# Autodesk Inventor assembly: Connector Box
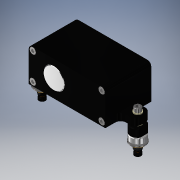
[picture p0: Inventor's stored thumbnail of the model, 180x180]
Saved by Autodesk Inventor 2019 (Build 230136000, 136)
## iProperties
Created: 2018-05-06
Part Number: Connector Box
Document SubType Name: Assembly
Designer: IEUser
Author: IEUser
## Documents named in this file (11)
- C:\Users\IEUser\Desktop\lrut-inflatable-ring-standard-master\Connector Box\Connector Box.iam
- C:\Users\IEUser\Desktop\lrut-inflatable-ring-standard-master\Connector Box\Connector Lid.ipt
- C:\Users\IEUser\Desktop\lrut-inflatable-ring-standard-master\Stock Components\LEMO\73397830-9-egg_4b_324_cll\egg_4b_324_cll_01.ipt
- C:\Users\IEUser\Desktop\lrut-inflatable-ring-standard-master\Stock Components\LEMO\73397830-9-egg_4b_324_cll\egg_4b_324_cll_02.ipt
- C:\Users\IEUser\Desktop\lrut-inflatable-ring-standard-master\Stock Components\LEMO\73397830-9-egg_4b_324_cll\egg_4b_324_cll_03.ipt
- C:\Users\IEUser\Desktop\lrut-inflatable-ring-standard-master\Connector Box\Connector Box.ipt
- C:\Users\IEUser\Desktop\lrut-inflatable-ring-standard-master\Stock Components\Accu Group\SSCF-M5-10-A4.ipt
- C:\Users\IEUser\Desktop\lrut-inflatable-ring-standard-master\Stock Components\Accu Group\HSHW-M5-6.6-N.ipt
- C:\Users\IEUser\Desktop\lrut-inflatable-ring-standard-master\Stock Components\Accu Group\HPW-5.2-10-3-N.ipt
- C:\Users\IEUser\Desktop\lrut-inflatable-ring-standard-master\Stock Components\Accu Group\SSCF-M5-20-A4.ipt
- C:\Users\IEUser\Desktop\lrut-inflatable-ring-standard-master\Spigots\Spigot Long.iam
## Components (17 placed, 10 different names)
1. Connector Lid:1 — Insert:1, Insert:2, Mate:1, Mate:2, Mate:3, Insert:4, Insert:5, Insert:6, Insert:7
2. egg_4b_324_cll_01:1 — Insert:1
3. egg_4b_324_cll_02:1 — Insert:2, Insert:3
4. egg_4b_324_cll_03:1 — Insert:3
5. Connector Box:1 — Mate:1, Mate:2, Mate:3, Insert:8, Insert:9, Insert:10, Insert:11, Angle:1, Angle:2
6. SSCF-M5-10-A4:1 — Insert:4
7. SSCF-M5-10-A4:2 — Insert:5
8. SSCF-M5-10-A4:3 — Insert:6
9. SSCF-M5-10-A4:4 — Insert:7
10. HSHW-M5-6.6-N:1 — Insert:8, Insert:12
11. HSHW-M5-6.6-N:2 — Insert:9, Insert:13
12. HPW-5.2-10-3-N:1 — Insert:10, Insert:14
13. HPW-5.2-10-3-N:2 — Insert:11, Insert:15
14. SSCF-M5-20-A4:1 — Insert:12
15. SSCF-M5-20-A4:2 — Insert:13
16. Spigot Long:1 [sub-assembly] — Insert:14, Angle:1
17. Spigot Long:2 [sub-assembly] — Insert:15, Angle:2
## Relationships (20: Insert 15, Mate 3, Angle 2)
- Insert:1: Connector Lid:1 ↔ egg_4b_324_cll_01:1
- Insert:2 (0.35 mm): Connector Lid:1 ↔ egg_4b_324_cll_02:1
- Insert:3 (0.35 mm): egg_4b_324_cll_02:1 ↔ egg_4b_324_cll_03:1
- Mate:1: Connector Lid:1 ↔ Connector Box:1
- Mate:2: Connector Lid:1 ↔ Connector Box:1
- Mate:3: Connector Lid:1 ↔ Connector Box:1
- Insert:4: Connector Lid:1 ↔ SSCF-M5-10-A4:1
- Insert:5: Connector Lid:1 ↔ SSCF-M5-10-A4:2
- Insert:6: Connector Lid:1 ↔ SSCF-M5-10-A4:3
- Insert:7: Connector Lid:1 ↔ SSCF-M5-10-A4:4
- Insert:8: Connector Box:1 ↔ HSHW-M5-6.6-N:1
- Insert:9: Connector Box:1 ↔ HSHW-M5-6.6-N:2
- Insert:10: Connector Box:1 ↔ HPW-5.2-10-3-N:1
- Insert:11: Connector Box:1 ↔ HPW-5.2-10-3-N:2
- Insert:12: HSHW-M5-6.6-N:1 ↔ SSCF-M5-20-A4:1
- Insert:13: HSHW-M5-6.6-N:2 ↔ SSCF-M5-20-A4:2
- Insert:14: HPW-5.2-10-3-N:1 ↔ Spigot Long:1
- Insert:15: HPW-5.2-10-3-N:2 ↔ Spigot Long:2
- Angle:1 (0 deg): Connector Box:1 ↔ Spigot Long:1
- Angle:2 (0 deg): Connector Box:1 ↔ Spigot Long:2
